# Autodesk Inventor assembly: ASSY_HGB_80-1
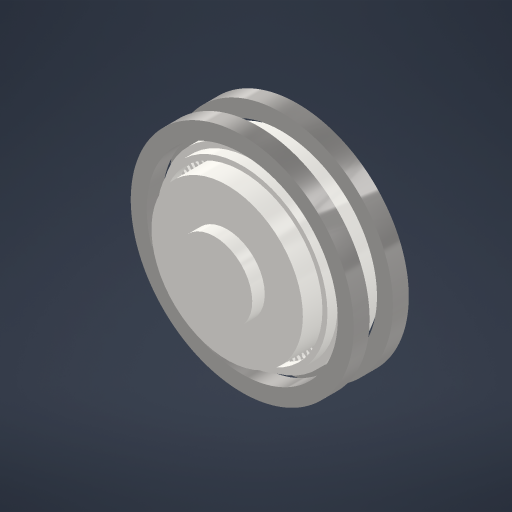
[picture p0: Inventor's stored thumbnail of the model, 512x512]
Saved by Autodesk Inventor 2024.2 (Build 282272000, 272)
## iProperties
Created: 2026-01-16
Part Number: ASSY_HGB_80-1
Document SubType Name: Assembly
Designer: 4aida
Author: 4aida
## Documents named in this file (5)
- C:\Users\4aida\OneDrive\Documents\CADING\DESIGN FILES\STANDARDS\Harmonic_GB\ASSY_HGB_80-1.iam
- C:\Users\4aida\OneDrive\Documents\CADING\DESIGN FILES\STANDARDS\Harmonic_GB\OUTER_GEAR_HGB.iam
- C:\Users\4aida\OneDrive\Documents\CADING\DESIGN FILES\STANDARDS\Harmonic_GB\INNER_GEAR_HGB.iam
- C:\Users\4aida\OneDrive\Documents\CADING\DESIGN FILES\STANDARDS\Harmonic_GB\BEARING_HGB.ipt
- C:\Users\4aida\OneDrive\Documents\CADING\DESIGN FILES\STANDARDS\Harmonic_GB\HARMONIC_GB.xlsx
## Components (4 placed, 3 different names)
1. OUTER_GEAR_HGB:1 [sub-assembly] — Mate:1, Mate:2, Angle:1, Mate:3, Flush:1, Mate:4, Mate:5, Flush:2, Flush:3
2. INNER_GEAR_HGB:1 [sub-assembly] — Mate:3, Flush:1
3. BEARING_HGB:1 — Mate:4, Flush:2
4. BEARING_HGB:2 — Mate:5, Flush:3
## Relationships (9: Mate 5, Flush 3, Angle 1)
- Mate:1: OUTER_GEAR_HGB:1
- Mate:2: OUTER_GEAR_HGB:1
- Angle:1 (0 deg): OUTER_GEAR_HGB:1
- Mate:3: OUTER_GEAR_HGB:1 ↔ INNER_GEAR_HGB:1
- Flush:1: OUTER_GEAR_HGB:1 ↔ INNER_GEAR_HGB:1
- Mate:4: OUTER_GEAR_HGB:1 ↔ BEARING_HGB:1
- Mate:5: OUTER_GEAR_HGB:1 ↔ BEARING_HGB:2
- Flush:2: OUTER_GEAR_HGB:1 ↔ BEARING_HGB:1
- Flush:3: OUTER_GEAR_HGB:1 ↔ BEARING_HGB:2
## Named parameters: N_ = 80, DP_ = 0.8 mm, OD_ = 60 mm, t_ = 3 mm, h_ = 30 mm, f_ = 5 mm
